# Autodesk Inventor assembly: Horizontal Shooter 1.1
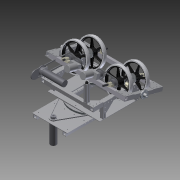
[picture p0: Inventor's stored thumbnail of the model, 180x180]
Saved by Autodesk Inventor 2011 SP1 (Build 150282100, 282)
## iProperties
Created: 2012-01-20
Part Number: Horizontal Shooter 1.1
Document SubType Name: Assembly
Designer: Christopher
Author: Christopher
## Documents named in this file (32)
- C:\Users\Christopher\Documents\Christopher\FIRST\Inventor files\2012\Horizontal Shooter 1\Horizontal Shooter 1.1.iam
- C:\Users\Christopher\Documents\Christopher\FIRST\Inventor files\2012\shooter design 2\10 inch side piece.ipt
- C:\Users\Christopher\Documents\Christopher\FIRST\Inventor files\2011\Kit of Parts\Chassis\Chassis_Wheel_AndyMark_am-0420.iam
- C:\Users\Christopher\Documents\Christopher\FIRST\Inventor files\2012\shooter design 2\wheel hub.ipt
- C:\Users\Christopher\Documents\Christopher\FIRST\Inventor files\2012\shooter design 2\proxybearing.ipt
- C:\Users\Christopher\Documents\Christopher\FIRST\Inventor files\2012\shooter design 2\14 in axle.ipt
- C:\Users\Christopher\Documents\Christopher\FIRST\Inventor files\2012\shooter design 2\shooter 9 inch horizontal.ipt
- C:\Users\Christopher\Documents\Christopher\FIRST\Inventor files\2012\tower bottom second design\proxycimulator775.ipt
- C:\Users\Christopher\Documents\Christopher\FIRST\Inventor files\2012\4 wheel kicker version 1\proxy 775 motor.ipt
- C:\Users\Christopher\Documents\Christopher\FIRST\Inventor files\2012\tower bottom second design\2.5ingear proxy.ipt
- C:\Users\Christopher\Documents\Christopher\FIRST\Inventor files\2012\shooter design 2\shooterchain.ipt
- C:\Users\Christopher\Documents\Christopher\FIRST\Inventor files\2012\shooter design 2\12 inch middle piece.ipt
- C:\Users\Christopher\Documents\Christopher\FIRST\Inventor files\2012\shooter design 2\gearmotor proxy.ipt
- C:\Users\Christopher\Documents\Christopher\FIRST\Inventor files\2012\shooter design 2\gearmotor mounting plate.ipt
- C:\Users\Christopher\Documents\Christopher\FIRST\Inventor files\2012\shooter design 2\4.25 inch axle for shooter.ipt
- C:\Users\Christopher\Documents\Christopher\FIRST\Inventor files\2012\shooter design 2\shooter elevation change proxy chain.ipt
- C:\Users\Christopher\Documents\Christopher\FIRST\Inventor files\2012\shooter design 2\5 in shooter standoff.ipt
- C:\Users\Christopher\Documents\Christopher\FIRST\Inventor files\2012\tower first design\doorstop.ipt
- C:\Users\Christopher\Documents\Christopher\FIRST\Inventor files\2012\rotating turret\inner piece.ipt
- C:\Users\Christopher\Documents\Christopher\FIRST\Inventor files\2012\rotating turret\outer piece.ipt
- C:\Users\Christopher\Documents\Christopher\FIRST\Inventor files\2012\rotating turret\top plate.ipt
- C:\Users\Christopher\Documents\Christopher\FIRST\Inventor files\2012\rotating turret\10 in tube.ipt
- C:\Users\Christopher\Documents\Christopher\FIRST\Inventor files\2012\rotating turret\12 in tube.ipt
- C:\Users\Christopher\Documents\Christopher\FIRST\Inventor files\2012\rotating turret\bottom plate.ipt
- C:\Users\Christopher\Documents\Christopher\FIRST\Inventor files\2012\rotating turret\smaller gear.ipt
- C:\Users\Christopher\Documents\Christopher\FIRST\Inventor files\2012\rotating turret\neck chain 1.1.ipt
- C:\Users\Christopher\Documents\Christopher\FIRST\Inventor files\2012\rotating turret\middle-top spacer plate.ipt
- C:\Users\Christopher\Documents\Christopher\FIRST\Inventor files\2012\shooter design 2\common angle bracket.ipt
- C:\Users\Christopher\Documents\Christopher\FIRST\Inventor files\2012\shooter design 2\motor stop for turret.ipt
- C:\Users\Christopher\Documents\Christopher\FIRST\Inventor files\2012\shooter design 2\shooterchain2.ipt
- C:\Users\Christopher\Documents\Christopher\FIRST\Inventor files\2012\Horizontal Shooter 1\new horizontall kicker thing.ipt
- C:\Users\Christopher\Documents\Christopher\FIRST\Inventor files\2012\Horizontal Shooter 1\new horizontal kicker thingleft.ipt
## Components (83 placed, 31 different names)
1. 10 inch side piece:1 — Flush:14, Flush:15, Mate:7, Mate:26, Flush:48, Flush:49, Mate:28, Flush:54, Mate:62, Mate:65, Flush:90, Flush:91, Flush:96, Insert:44, Insert:45, Insert:53, Insert:55, Insert:56, Flush:111, Insert:57
2. 10 inch side piece:2 — Mate:8, Flush:16, Flush:17, Flush:52, Flush:53, Mate:27, Mate:59, Flush:84, Flush:85, Flush:94, Insert:43, Flush:98, Mate:70, Flush:101, Insert:46, Insert:47, Insert:50, Insert:51, Insert:54
3. Chassis_Wheel_AndyMark_am-0420:1 [sub-assembly] — Insert:1
4. Chassis_Wheel_AndyMark_am-0420:2 [sub-assembly] — Insert:2
5. Chassis_Wheel_AndyMark_am-0420:3 [sub-assembly] — Insert:3
6. Chassis_Wheel_AndyMark_am-0420:4 [sub-assembly] — Insert:4
7. wheel hub:1 — Insert:1, Insert:10
8. wheel hub:2 — Insert:2, Insert:9
9. wheel hub:3 — Insert:3, Insert:11
10. wheel hub:4 — Insert:4, Insert:12
11. proxybearing:1 — Insert:8, Insert:17, Flush:125
12. proxybearing:2 — Mate:8, Flush:16, Flush:17, Insert:31
13. proxybearing:3 — Insert:7, Insert:79, Mate:72, Flush:122
14. proxybearing:4 — Insert:6, Mate:31, Flush:126
15. proxybearing:5 — Flush:14, Flush:15, Mate:7, Insert:97
16. proxybearing:6 — Insert:5, Flush:38, Mate:31, Flush:127, Mate:74
17. 14 in axle:1 — Insert:6, Insert:7, Insert:11, Insert:12
18. 14 in axle:2 — Insert:5, Insert:8, Insert:9, Insert:10
19. shooter 9 inch horizontal:1 — Flush:38, Insert:62, Insert:64, Insert:65, Insert:75, Flush:119, Flush:121, Insert:91, Insert:92
20. shooter 9 inch horizontal:2 — Flush:116, Insert:81, Insert:82, Insert:83, Insert:84, Flush:120, Insert:94, Insert:95
21. proxycimulator775:1 — Insert:77, Insert:78, Flush:116, Flush:123
22. proxycimulator775:2 — Insert:14, Insert:18, Flush:124, Mate:73
23. proxy 775 motor:1 — Insert:77
24. proxy 775 motor:2 — Insert:14
25. 2.5ingear proxy:1 — Insert:78, Insert:80
26. 2.5ingear proxy:2 — Insert:79, Insert:87
27. 2.5ingear proxy:3 — Insert:18, Insert:20
28. 2.5ingear proxy:4 — Insert:17, Insert:85
29. shooterchain:2 — Insert:20, Insert:85
30. wheel hub:5 — Insert:91, Insert:92, Insert:96
31. wheel hub:6 — Insert:94, Insert:95
32. 12 inch middle piece:1 — Mate:26, Flush:48, Flush:49, Flush:52, Flush:53, Mate:27, Flush:55, Insert:48, Insert:49, Insert:52, Insert:58, Flush:112
33. gearmotor proxy:1 — Insert:33
34. gearmotor mounting plate:1 — Mate:28, Flush:54, Flush:55, Insert:98
35. 4.25 inch axle for shooter:1 — Insert:31, Insert:96
36. 2.5ingear proxy:5 — Insert:35, Insert:97
37. 2.5ingear proxy:6 — Insert:33, Insert:98
38. shooter elevation change proxy chain:1 — Insert:35
39. doorstop:1 — Insert:60
40. 5 in shooter standoff:2 — Mate:58, Mate:59, Flush:84, Flush:85, Flush:87, Mate:60, Flush:94, Flush:105, Flush:109
41. 5 in shooter standoff:4 — Mate:62, Mate:63, Flush:88, Flush:89, Flush:100, Flush:106, Flush:110
42. 5 in shooter standoff:5 — Mate:64, Mate:65, Flush:90, Flush:91, Mate:66, Flush:92, Flush:96, Flush:99, Flush:107
43. inner piece:1 — Insert:36, Insert:37, Insert:38
44. outer piece:1 — Insert:36, Tangent:3, Tangent:4, Mate:56
45. top plate:1 — Tangent:3, Tangent:4, Mate:55, Flush:78, Flush:79, Mate:58, Flush:86, Mate:63, Flush:88, Flush:89, Mate:64, Mate:67, Mate:69, Flush:103, Flush:104, Flush:105, Flush:106, Flush:107
46. 10 in tube:1 — Flush:66, Mate:39, Flush:67, Mate:52
47. 12 in tube:1 — Flush:66, Mate:39, Flush:67, Mate:41, Flush:70, Flush:71, Flush:73, Flush:77, Mate:54
48. 10 in tube:2 — Mate:41, Flush:70, Flush:71, Flush:72
49. 12 in tube:2 — Mate:52, Flush:77, Mate:53
50. bottom plate:1 — Flush:72, Flush:73, Insert:37, Insert:38, Insert:39, Insert:40, Mate:53, Mate:54
51. 5 in shooter standoff:6 — Flush:86, Flush:87, Mate:60, Mate:61, Tangent:11, Tangent:12
52. 5 in shooter standoff:7 — Mate:66, Flush:92, Mate:67, Mate:68, Tangent:13, Tangent:14
53. doorstop:2 — Mate:68, Tangent:13, Tangent:14
54. doorstop:3 — Mate:61, Tangent:11, Tangent:12
55. gearmotor proxy:2 — Insert:39
56. smaller gear:1 — Insert:40, Insert:41
57. neck chain 1.1:1 — Insert:41
58. middle-top spacer plate:1 — Mate:55, Flush:78, Flush:79, Mate:56
59. common angle bracket:2 — Insert:44, Flush:99
60. common angle bracket:3 — Insert:45, Flush:100
61. common angle bracket:4 — Insert:43, Flush:98
62. common angle bracket:5 — Insert:46, Flush:102
63. 5 in shooter standoff:8 — Mate:69, Mate:70, Flush:101, Flush:102, Flush:103, Flush:104, Flush:108
64. common angle bracket:6 — Insert:51, Flush:108
65. common angle bracket:7 — Insert:47, Insert:48, Insert:59
66. common angle bracket:8 — Insert:54, Flush:109
67. common angle bracket:9 — Insert:49, Insert:50
68. common angle bracket:10 — Insert:52, Insert:53
69. common angle bracket:11 — Insert:56, Flush:111
70. common angle bracket:12 — Insert:57, Insert:58
71. common angle bracket:13 — Insert:55, Flush:110
72. motor stop for turret:1 — Insert:59, Flush:112, Insert:60
73. common angle bracket:14 — Insert:83, Insert:90
74. common angle bracket:15 — Insert:81, Insert:88
75. common angle bracket:16 — Insert:65, Insert:93
76. common angle bracket:17 — Insert:62, Insert:86
77. common angle bracket:18 — Insert:64
78. common angle bracket:19 — Insert:75, Insert:89
79. common angle bracket:20 — Insert:82
80. common angle bracket:21 — Insert:84, Mate:71
81. shooterchain2:1 — Insert:80, Insert:87
82. new horizontall kicker thing:1 — Insert:86, Flush:119, Insert:88, Flush:126, Flush:127, Mate:74
83. new horizontal kicker thingleft:1 — Flush:120, Mate:71, Flush:121, Insert:89, Insert:90, Mate:72, Flush:122, Flush:123, Flush:124, Flush:125, Mate:73, Insert:93
## Relationships (161: Insert 69, Flush 56, Mate 30, Tangent 6)
- Insert:1: Chassis_Wheel_AndyMark_am-0420:1 ↔ wheel hub:1
- Insert:2: Chassis_Wheel_AndyMark_am-0420:2 ↔ wheel hub:2
- Insert:3: Chassis_Wheel_AndyMark_am-0420:3 ↔ wheel hub:3
- Insert:4: Chassis_Wheel_AndyMark_am-0420:4 ↔ wheel hub:4
- Flush:14: 10 inch side piece:1 ↔ proxybearing:5
- Flush:15 (50.8 mm): 10 inch side piece:1 ↔ proxybearing:5
- Mate:7: 10 inch side piece:1 ↔ proxybearing:5
- Mate:8: 10 inch side piece:2 ↔ proxybearing:2
- Flush:16: 10 inch side piece:2 ↔ proxybearing:2
- Flush:17 (50.8 mm): 10 inch side piece:2 ↔ proxybearing:2
- Insert:5 (-12.7 mm): proxybearing:6 ↔ 14 in axle:2
- Insert:6 (-38.1 mm): proxybearing:4 ↔ 14 in axle:1
- Flush:38 (-114.3 mm): proxybearing:6 ↔ shooter 9 inch horizontal:1
- Insert:7 (12.7 mm): proxybearing:3 ↔ 14 in axle:1
- Insert:8 (38.1 mm): proxybearing:1 ↔ 14 in axle:2
- Insert:9 (117.475 mm): wheel hub:2 ↔ 14 in axle:2
- Insert:10 (142.875 mm): wheel hub:1 ↔ 14 in axle:2
- Insert:11 (142.875 mm): wheel hub:3 ↔ 14 in axle:1
- Insert:12 (117.475 mm): wheel hub:4 ↔ 14 in axle:1
- Insert:14: proxycimulator775:2 ↔ proxy 775 motor:2
- Insert:17: proxybearing:1 ↔ 2.5ingear proxy:4
- Insert:18: proxycimulator775:2 ↔ 2.5ingear proxy:3
- Insert:20: 2.5ingear proxy:3 ↔ shooterchain:2
- Mate:26: 10 inch side piece:1 ↔ 12 inch middle piece:1
- Flush:48: 10 inch side piece:1 ↔ 12 inch middle piece:1
- Flush:49: 10 inch side piece:1 ↔ 12 inch middle piece:1
- Flush:52: 10 inch side piece:2 ↔ 12 inch middle piece:1
- Flush:53: 10 inch side piece:2 ↔ 12 inch middle piece:1
- Mate:27: 10 inch side piece:2 ↔ 12 inch middle piece:1
- Mate:28: 10 inch side piece:1 ↔ gearmotor mounting plate:1
- Flush:54: 10 inch side piece:1 ↔ gearmotor mounting plate:1
- Flush:55: 12 inch middle piece:1 ↔ gearmotor mounting plate:1
- Insert:31 (-25.4 mm): proxybearing:2 ↔ 4.25 inch axle for shooter:1
- Insert:33: gearmotor proxy:1 ↔ 2.5ingear proxy:6
- Insert:35: 2.5ingear proxy:5 ↔ shooter elevation change proxy chain:1
- Mate:31 (285.75 mm): proxybearing:4 ↔ proxybearing:6
- Insert:36: inner piece:1 ↔ outer piece:1
- Flush:66: 10 in tube:1 ↔ 12 in tube:1
- Mate:39: 10 in tube:1 ↔ 12 in tube:1
- Flush:67 (139.7 mm): 10 in tube:1 ↔ 12 in tube:1
- Mate:41: 12 in tube:1 ↔ 10 in tube:2
- Flush:70: 12 in tube:1 ↔ 10 in tube:2
- Flush:71: 12 in tube:1 ↔ 10 in tube:2
- Flush:72: 10 in tube:2 ↔ bottom plate:1
- Flush:73 (9.525 mm): 12 in tube:1 ↔ bottom plate:1
- Insert:37: inner piece:1 ↔ bottom plate:1
- Insert:38: inner piece:1 ↔ bottom plate:1
- Tangent:3: outer piece:1 ↔ top plate:1
- Tangent:4 (41.275 mm): outer piece:1 ↔ top plate:1
- Insert:39: bottom plate:1 ↔ gearmotor proxy:2
- Insert:40: bottom plate:1 ↔ smaller gear:1
- Insert:41: smaller gear:1 ↔ neck chain 1.1:1
- Mate:52: 10 in tube:1 ↔ 12 in tube:2
- Flush:77: 12 in tube:1 ↔ 12 in tube:2
- Mate:53: 12 in tube:2 ↔ bottom plate:1
- Mate:54: 12 in tube:1 ↔ bottom plate:1
- Mate:55: top plate:1 ↔ middle-top spacer plate:1
- Flush:78: top plate:1 ↔ middle-top spacer plate:1
- Flush:79: top plate:1 ↔ middle-top spacer plate:1
- Mate:56: outer piece:1 ↔ middle-top spacer plate:1
- Mate:58: 5 in shooter standoff:2 ↔ top plate:1
- Mate:59: 10 inch side piece:2 ↔ 5 in shooter standoff:2
- Flush:84: 10 inch side piece:2 ↔ 5 in shooter standoff:2
- Flush:85: 10 inch side piece:2 ↔ 5 in shooter standoff:2
- Flush:86 (28.575 mm): top plate:1 ↔ 5 in shooter standoff:6
- Flush:87: 5 in shooter standoff:2 ↔ 5 in shooter standoff:6
- Mate:60: 5 in shooter standoff:2 ↔ 5 in shooter standoff:6
- Mate:61: 5 in shooter standoff:6 ↔ doorstop:3
- Tangent:11: 5 in shooter standoff:6 ↔ doorstop:3
- Tangent:12 (22.225 mm): 5 in shooter standoff:6 ↔ doorstop:3
- Mate:62: 10 inch side piece:1 ↔ 5 in shooter standoff:4
- Mate:63: 5 in shooter standoff:4 ↔ top plate:1
- Flush:88: 5 in shooter standoff:4 ↔ top plate:1
- Flush:89 (-25.4 mm): 5 in shooter standoff:4 ↔ top plate:1
- Mate:64: 5 in shooter standoff:5 ↔ top plate:1
- Mate:65: 10 inch side piece:1 ↔ 5 in shooter standoff:5
- Flush:90: 10 inch side piece:1 ↔ 5 in shooter standoff:5
- Flush:91: 10 inch side piece:1 ↔ 5 in shooter standoff:5
- Mate:66: 5 in shooter standoff:5 ↔ 5 in shooter standoff:7
- Flush:92: 5 in shooter standoff:5 ↔ 5 in shooter standoff:7
- Mate:67 (25.4 mm): top plate:1 ↔ 5 in shooter standoff:7
- Mate:68: 5 in shooter standoff:7 ↔ doorstop:2
- Tangent:13 (-28.575 mm): 5 in shooter standoff:7 ↔ doorstop:2
- Tangent:14 (-15.875 mm): 5 in shooter standoff:7 ↔ doorstop:2
- Flush:94: 10 inch side piece:2 ↔ 5 in shooter standoff:2
- Flush:96: 10 inch side piece:1 ↔ 5 in shooter standoff:5
- Insert:43: 10 inch side piece:2 ↔ common angle bracket:4
- Flush:98: 10 inch side piece:2 ↔ common angle bracket:4
- Insert:44: 10 inch side piece:1 ↔ common angle bracket:2
- Flush:99: 5 in shooter standoff:5 ↔ common angle bracket:2
- Insert:45: 10 inch side piece:1 ↔ common angle bracket:3
- Flush:100: 5 in shooter standoff:4 ↔ common angle bracket:3
- Mate:69: top plate:1 ↔ 5 in shooter standoff:8
- Mate:70: 10 inch side piece:2 ↔ 5 in shooter standoff:8
- Flush:101: 10 inch side piece:2 ↔ 5 in shooter standoff:8
- Insert:46: 10 inch side piece:2 ↔ common angle bracket:5
- Flush:102: common angle bracket:5 ↔ 5 in shooter standoff:8
- Flush:103 (25.4 mm): top plate:1 ↔ 5 in shooter standoff:8
- Flush:104: top plate:1 ↔ 5 in shooter standoff:8
- Flush:105: 5 in shooter standoff:2 ↔ top plate:1
- Flush:106: 5 in shooter standoff:4 ↔ top plate:1
- Flush:107: 5 in shooter standoff:5 ↔ top plate:1
- Insert:47: 10 inch side piece:2 ↔ common angle bracket:7
- Insert:48: 12 inch middle piece:1 ↔ common angle bracket:7
- Insert:49: 12 inch middle piece:1 ↔ common angle bracket:9
- Insert:50: 10 inch side piece:2 ↔ common angle bracket:9
- Insert:51: 10 inch side piece:2 ↔ common angle bracket:6
- Insert:52: 12 inch middle piece:1 ↔ common angle bracket:10
- Insert:53: 10 inch side piece:1 ↔ common angle bracket:10
- Flush:108: 5 in shooter standoff:8 ↔ common angle bracket:6
- Insert:54: 10 inch side piece:2 ↔ common angle bracket:8
- Flush:109: 5 in shooter standoff:2 ↔ common angle bracket:8
- Insert:55: 10 inch side piece:1 ↔ common angle bracket:13
- Flush:110: 5 in shooter standoff:4 ↔ common angle bracket:13
- Insert:56: 10 inch side piece:1 ↔ common angle bracket:11
- Flush:111: 10 inch side piece:1 ↔ common angle bracket:11
- Insert:57: 10 inch side piece:1 ↔ common angle bracket:12
- Insert:58: 12 inch middle piece:1 ↔ common angle bracket:12
- Insert:59: common angle bracket:7 ↔ motor stop for turret:1
- Flush:112: 12 inch middle piece:1 ↔ motor stop for turret:1
- Insert:60: doorstop:1 ↔ motor stop for turret:1
- Insert:62: shooter 9 inch horizontal:1 ↔ common angle bracket:17
- Insert:64: shooter 9 inch horizontal:1 ↔ common angle bracket:18
- Insert:65: shooter 9 inch horizontal:1 ↔ common angle bracket:16
- Insert:75: shooter 9 inch horizontal:1 ↔ common angle bracket:19
- Insert:77: proxycimulator775:1 ↔ proxy 775 motor:1
- Insert:78: proxycimulator775:1 ↔ 2.5ingear proxy:1
- Flush:116 (177.8 mm): shooter 9 inch horizontal:2 ↔ proxycimulator775:1
- Insert:79: proxybearing:3 ↔ 2.5ingear proxy:2
- Insert:80: 2.5ingear proxy:1 ↔ shooterchain2:1
- Insert:81: shooter 9 inch horizontal:2 ↔ common angle bracket:15
- Insert:82: shooter 9 inch horizontal:2 ↔ common angle bracket:20
- Insert:83: shooter 9 inch horizontal:2 ↔ common angle bracket:14
- Insert:84: shooter 9 inch horizontal:2 ↔ common angle bracket:21
- Insert:85: 2.5ingear proxy:4 ↔ shooterchain:2
- Insert:86: common angle bracket:17 ↔ new horizontall kicker thing:1
- Insert:87: 2.5ingear proxy:2 ↔ shooterchain2:1
- Flush:119: shooter 9 inch horizontal:1 ↔ new horizontall kicker thing:1
- Insert:88: common angle bracket:15 ↔ new horizontall kicker thing:1
- Flush:120: shooter 9 inch horizontal:2 ↔ new horizontal kicker thingleft:1
- Mate:71: common angle bracket:21 ↔ new horizontal kicker thingleft:1
- Flush:121: shooter 9 inch horizontal:1 ↔ new horizontal kicker thingleft:1
- Insert:89: common angle bracket:19 ↔ new horizontal kicker thingleft:1
- Insert:90: common angle bracket:14 ↔ new horizontal kicker thingleft:1
- Mate:72: proxybearing:3 ↔ new horizontal kicker thingleft:1
- Flush:122: proxybearing:3 ↔ new horizontal kicker thingleft:1
- Flush:123: proxycimulator775:1 ↔ new horizontal kicker thingleft:1
- Flush:124: proxycimulator775:2 ↔ new horizontal kicker thingleft:1
- Flush:125: proxybearing:1 ↔ new horizontal kicker thingleft:1
- Flush:126: proxybearing:4 ↔ new horizontall kicker thing:1
- Flush:127: proxybearing:6 ↔ new horizontall kicker thing:1
- Insert:91: shooter 9 inch horizontal:1 ↔ wheel hub:5
- Insert:92: shooter 9 inch horizontal:1 ↔ wheel hub:5
- Mate:73: proxycimulator775:2 ↔ new horizontal kicker thingleft:1
- Insert:93: common angle bracket:16 ↔ new horizontal kicker thingleft:1
- Mate:74: proxybearing:6 ↔ new horizontall kicker thing:1
- Insert:94: shooter 9 inch horizontal:2 ↔ wheel hub:6
- Insert:95: shooter 9 inch horizontal:2 ↔ wheel hub:6
- Insert:96 (-114.3 mm): wheel hub:5 ↔ 4.25 inch axle for shooter:1
- Insert:97: proxybearing:5 ↔ 2.5ingear proxy:5
- Insert:98: gearmotor mounting plate:1 ↔ 2.5ingear proxy:6
